# Autodesk Inventor assembly: pihti-for-simulation
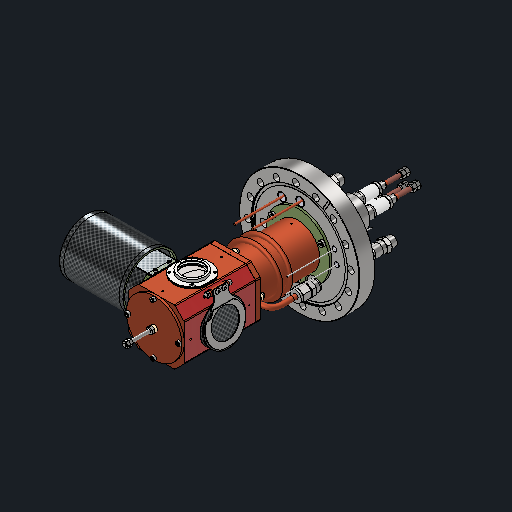
[picture p0: Inventor's stored thumbnail of the model, 512x512]
Saved by Autodesk Inventor 2027.1 (Build 311270010, 270A)
## iProperties
Created: 2024-05-09
Part Number: pihti-for-simulation
Document SubType Name: Assembly
Designer: kuzmin
Mass: 19614.5 g
Surface Area: 13609.5 cm^2
Volume: 3689.47 cm^3
Density: 5.31636 g/cm^3
Author: kuzmin
## Documents named in this file (10)
- C:\Users\queezz\Dropbox\Drawings\pihti-cad\Plasma Vessel\pihti-for-simulation.iam
- C:\Users\queezz\Dropbox\Drawings\pihti-cad\Plasma Vessel\Plasma-Flange-2024\cathode-box-on-a-flange.iam
- C:\Users\queezz\Dropbox\Drawings\pihti-cad\Plasma Vessel\Cathode-Anode-Flange\Cathode-Anode-70IC-flange-with-feeds.iam
- C:\Users\queezz\Dropbox\Drawings\pihti-cad\Plasma Vessel\Plasma-Box\Plasma-box-hayashi-aka-upgrade.iam
- C:\Users\queezz\Dropbox\Drawings\pihti-cad\ContentCenter\Fastners\M3x8-SHCS.ipt
- C:\Users\queezz\Dropbox\Drawings\pihti-cad\Plasma Vessel\Plasma-Box\probe-gate-with-spindel.iam
- C:\Users\queezz\Dropbox\Drawings\pihti-cad\Plasma Vessel\Cathode-Anode-Flange\cf70_spacer.ipt
- C:\Users\queezz\Dropbox\Drawings\pihti-cad\Plasma Vessel\Plasma-Box\anode-on-flange.iam
- C:\Users\queezz\Dropbox\Drawings\pihti-cad\Plasma Vessel\entrance-mesh-assembly.iam
- C:\Users\queezz\Dropbox\Drawings\pihti-cad\Plasma Vessel\probe-port-mesh-welded.iam
## Components (16 placed, 9 different names)
1. cathode-box-on-a-flange:1 [sub-assembly] — Mate:2, Mate:5, Rigid:10
2. Cathode-Anode-70IC-flange-with-feeds:1 [sub-assembly] — Mate:2, Mate:5, Mate:6
3. Plasma-box-hayashi-aka-upgrade:1 [sub-assembly] — Mate:3, Mate:4, Hinge Angle, Mate:7, Mate:8, Mate:9, Mate:13, Mate:17
4. probe-gate-with-spindel:1 [sub-assembly] — Mate:3, Mate:4, Hinge Angle
5. cf70_spacer:1 — Rigid:10, Mate:6
6. anode-on-flange:1 [sub-assembly] — Mate:7, Mate:8, Mate:9, Rigid:11, Rigid:12, Rigid:13, Rigid:14
7. entrance-mesh-assembly:1 [sub-assembly] — Mate:13, Mate:17, Mate:19
8. probe-port-mesh-welded:1 [sub-assembly] — Mate:19
9. SS ISO 4762 M3 x 8:5 — Rigid:11
10. SS ISO 4762 M3 x 8:6 — Rigid:12
11. SS ISO 4762 M3 x 8:7 — Rigid:14
12. SS ISO 4762 M3 x 8:8 — Rigid:13
13. SS ISO 4762 M3 x 8:1
14. SS ISO 4762 M3 x 8:2
15. SS ISO 4762 M3 x 8:3
16. SS ISO 4762 M3 x 8:4
## Relationships (17: Mate 11, WeldJoint 5, Angle 1)
- Mate:2: cathode-box-on-a-flange:1 ↔ Cathode-Anode-70IC-flange-with-feeds:1
- Mate:3: Plasma-box-hayashi-aka-upgrade:1 ↔ probe-gate-with-spindel:1
- Mate:4: Plasma-box-hayashi-aka-upgrade:1 ↔ probe-gate-with-spindel:1
- Hinge Angle [Angle] (45 deg): Plasma-box-hayashi-aka-upgrade:1 ↔ probe-gate-with-spindel:1
- Mate:5: cathode-box-on-a-flange:1 ↔ Cathode-Anode-70IC-flange-with-feeds:1
- Rigid:10 [WeldJoint]: cathode-box-on-a-flange:1 ↔ cf70_spacer:1
- Mate:6: Cathode-Anode-70IC-flange-with-feeds:1 ↔ cf70_spacer:1
- Mate:7: Plasma-box-hayashi-aka-upgrade:1 ↔ anode-on-flange:1
- Mate:8: Plasma-box-hayashi-aka-upgrade:1 ↔ anode-on-flange:1
- Mate:9: Plasma-box-hayashi-aka-upgrade:1 ↔ anode-on-flange:1
- Rigid:11 [WeldJoint]: anode-on-flange:1 ↔ SS ISO 4762 M3 x 8:5
- Rigid:12 [WeldJoint]: anode-on-flange:1 ↔ SS ISO 4762 M3 x 8:6
- Rigid:13 [WeldJoint]: anode-on-flange:1 ↔ SS ISO 4762 M3 x 8:8
- Rigid:14 [WeldJoint]: anode-on-flange:1 ↔ SS ISO 4762 M3 x 8:7
- Mate:13: Plasma-box-hayashi-aka-upgrade:1 ↔ entrance-mesh-assembly:1
- Mate:17: Plasma-box-hayashi-aka-upgrade:1 ↔ entrance-mesh-assembly:1
- Mate:19: entrance-mesh-assembly:1 ↔ probe-port-mesh-welded:1
